# Autodesk Inventor assembly: BatteryPack
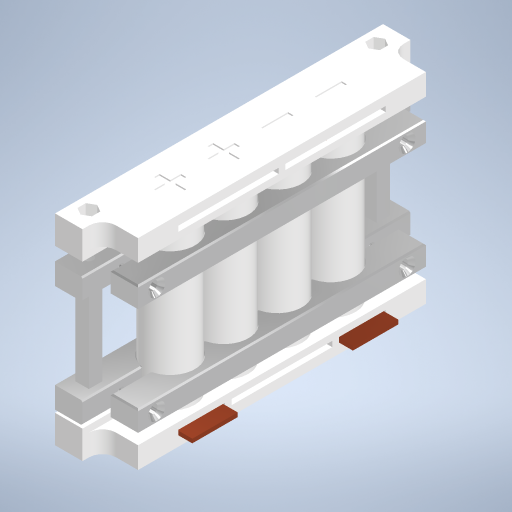
[picture p0: Inventor's stored thumbnail of the model, 512x512]
Saved by Autodesk Inventor 2023 (Build 270158000, 158)
## iProperties
Created: 2022-08-09
Part Number: BatteryPack
Document SubType Name: Assembly
Designer: Aditya Bansal
Author: Aditya Bansal
## Documents named in this file (9)
- C:\Users\Aditya Bansal\OneDrive - UNSW\Uni\BlueSat\rocketry-datasat\Structure\Electronics_Structure\Battery_V1\BatteryPack.iam
- C:\Users\Aditya Bansal\OneDrive - UNSW\Uni\BlueSat\rocketry-datasat\Structure\Electronics_Structure\Battery_V1\BatteryHolderTop.ipt
- C:\Users\Aditya Bansal\OneDrive - UNSW\Uni\BlueSat\rocketry-datasat\Structure\Electronics_Structure\Battery_V1\BatteryHolderBottom.ipt
- C:\Users\Aditya Bansal\OneDrive - UNSW\Uni\BlueSat\rocketry-datasat\Structure\Electronics_Structure\COTS\Battery_Cell_18650.ipt
- C:\Users\Aditya Bansal\OneDrive - UNSW\Uni\BlueSat\rocketry-datasat\Structure\Electronics_Structure\Battery_V1\BatteryStandoff.ipt
- C:\Users\Aditya Bansal\OneDrive - UNSW\Uni\BlueSat\rocketry-datasat\Structure\Electronics_Structure\Battery_V1\BatteryHolderEnd.ipt
- C:\Users\Aditya Bansal\OneDrive - UNSW\Uni\BlueSat\rocketry-datasat\Structure\Electronics_Structure\Battery_V1\BatteryHolderEndSeries.ipt
- C:\Users\Aditya Bansal\OneDrive - UNSW\Uni\BlueSat\rocketry-datasat\Structure\Electronics_Structure\Battery_V1\Tabs\LargeTab.ipt
- C:\Users\Aditya Bansal\OneDrive - UNSW\Uni\BlueSat\rocketry-datasat\Structure\Electronics_Structure\Battery_V1\Tabs\SmallTab.ipt
## Components (17 placed, 8 different names)
1. BatteryHolderBottom:1 — Mate:1, Mate:2, Mate:3, Mate:4, Mate:5, Mate:6, Mate:7, Mate:10, Mate:11, Mate:19, Mate:20, Mate:21, Mate:22, Mate:30
2. BatteryHolderTop:1 — Mate:8, Mate:9, Mate:10, Mate:11
3. Battery_Cell_18650:1 — Mate:4, Flush:2, Mate:8, Mate:17, Mate:24, Mate:27, Mate:47, Mate:48
4. Battery_Cell_18650:2 — Mate:1, Flush:1, Mate:9, Mate:16, Mate:18, Mate:25, Mate:26
5. Battery_Cell_18650:3 — Mate:2, Flush:1, Flush:3
6. Battery_Cell_18650:4 — Mate:3, Flush:2, Flush:3
7. BatteryHolderTop:2 — Mate:18
8. BatteryHolderBottom:2 — Mate:16, Mate:17, Mate:23
9. BatteryStandoff:1 — Mate:19, Mate:22, Mate:23
10. BatteryStandoff:2 — Mate:20, Mate:21
11. BatteryHolderEnd:1 — Mate:26, Mate:27, Mate:30, Mate:38, Mate:39, Mate:40, Mate:41, Mate:42, Mate:43, Mate:44, Mate:45, Mate:46
12. BatteryHolderEndSeries:1 — Mate:24, Mate:25, Mate:31, Mate:32, Mate:33, Mate:34, Mate:35, Mate:36
13. LargeTab:1 — Mate:31, Mate:32, Mate:33
14. LargeTab:2 — Mate:38, Mate:39, Mate:40
15. SmallTab:2 — Mate:44, Mate:45, Mate:46, Mate:47
16. LargeTab:3 — Mate:34, Mate:35, Mate:36, Mate:48
17. SmallTab:3 — Mate:41, Mate:42, Mate:43
## Relationships (46: Mate 43, Flush 3)
- Mate:1: BatteryHolderBottom:1 ↔ Battery_Cell_18650:2
- Mate:2: BatteryHolderBottom:1 ↔ Battery_Cell_18650:3
- Mate:3: BatteryHolderBottom:1 ↔ Battery_Cell_18650:4
- Mate:4: BatteryHolderBottom:1 ↔ Battery_Cell_18650:1
- Mate:5: BatteryHolderBottom:1
- Mate:6: BatteryHolderBottom:1
- Mate:7: BatteryHolderBottom:1
- Flush:1: Battery_Cell_18650:2 ↔ Battery_Cell_18650:3
- Flush:2: Battery_Cell_18650:1 ↔ Battery_Cell_18650:4
- Flush:3: Battery_Cell_18650:3 ↔ Battery_Cell_18650:4
- Mate:8: BatteryHolderTop:1 ↔ Battery_Cell_18650:1
- Mate:9: BatteryHolderTop:1 ↔ Battery_Cell_18650:2
- Mate:10: BatteryHolderBottom:1 ↔ BatteryHolderTop:1
- Mate:11: BatteryHolderBottom:1 ↔ BatteryHolderTop:1
- [Mate]: BatteryHolderTop:2 ↔ BatteryHolderBottom:2
- [Mate]: BatteryHolderTop:2 ↔ BatteryHolderBottom:2
- Mate:16: Battery_Cell_18650:2 ↔ BatteryHolderBottom:2
- Mate:17: Battery_Cell_18650:1 ↔ BatteryHolderBottom:2
- Mate:18: Battery_Cell_18650:2 ↔ BatteryHolderTop:2
- Mate:19: BatteryHolderBottom:1 ↔ BatteryStandoff:1
- Mate:20: BatteryHolderBottom:1 ↔ BatteryStandoff:2
- Mate:21: BatteryHolderBottom:1 ↔ BatteryStandoff:2
- Mate:22: BatteryHolderBottom:1 ↔ BatteryStandoff:1
- Mate:23: BatteryHolderBottom:2 ↔ BatteryStandoff:1
- Mate:24: Battery_Cell_18650:1 ↔ BatteryHolderEndSeries:1
- Mate:25: Battery_Cell_18650:2 ↔ BatteryHolderEndSeries:1
- Mate:26: Battery_Cell_18650:2 ↔ BatteryHolderEnd:1
- Mate:27: Battery_Cell_18650:1 ↔ BatteryHolderEnd:1
- Mate:30 (1 mm): BatteryHolderBottom:1 ↔ BatteryHolderEnd:1
- Mate:31: BatteryHolderEndSeries:1 ↔ LargeTab:1
- Mate:32: BatteryHolderEndSeries:1 ↔ LargeTab:1
- Mate:33 (0.25 mm): BatteryHolderEndSeries:1 ↔ LargeTab:1
- Mate:34: BatteryHolderEndSeries:1 ↔ LargeTab:3
- Mate:35: BatteryHolderEndSeries:1 ↔ LargeTab:3
- Mate:36 (0.25 mm): BatteryHolderEndSeries:1 ↔ LargeTab:3
- Mate:38: BatteryHolderEnd:1 ↔ LargeTab:2
- Mate:39 (0.25 mm): BatteryHolderEnd:1 ↔ LargeTab:2
- Mate:40: BatteryHolderEnd:1 ↔ LargeTab:2
- Mate:41: BatteryHolderEnd:1 ↔ SmallTab:3
- Mate:42: BatteryHolderEnd:1 ↔ SmallTab:3
- Mate:43 (0.25 mm): BatteryHolderEnd:1 ↔ SmallTab:3
- Mate:44: BatteryHolderEnd:1 ↔ SmallTab:2
- Mate:45: BatteryHolderEnd:1 ↔ SmallTab:2
- Mate:46 (0.25 mm): BatteryHolderEnd:1 ↔ SmallTab:2
- Mate:47: Battery_Cell_18650:1 ↔ SmallTab:2
- Mate:48: Battery_Cell_18650:1 ↔ LargeTab:3
## Named parameters: d15_d14 = 0 mm, d18_d13 = 0 mm
